# Autodesk Inventor assembly: TD6S-CHC_mockup
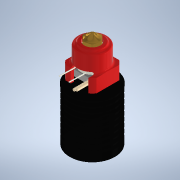
[picture p0: Inventor's stored thumbnail of the model, 180x180]
Saved by Autodesk Inventor 2020 (Build 240168000, 168)
## iProperties
Created: 2022-09-02
Part Number: TD6S-CHC_mockup
Description: STEP AP203
Document SubType Name: Assembly
Designer: Ishaan
Title: TD6S-CHC.STEP
Revision Number: ÈÎºÎ
## Documents named in this file (7)
- D:\Documents\Projects\Axiom - IDEX 3D Printer\CAD\00 - COTS Components\CHC Hotend\TD6S-CHC_mockup.iam
- D:\Documents\Projects\Axiom - IDEX 3D Printer\CAD\00 - COTS Components\CHC Hotend\Ã«Ï¸¹Üºí¹Ü×°Åä.iam
- D:\Documents\Projects\Axiom - IDEX 3D Printer\CAD\00 - COTS Components\CHC Hotend\»·ÐÎ¼ÓÈÈ¿é×°ÅäÌå1.iam
- D:\Documents\Projects\Axiom - IDEX 3D Printer\CAD\00 - COTS Components\CHC Hotend\socket head thin cap screw_din_DIN 7984 - M3 x 6 --- 4.5N.ipt
- D:\Documents\Projects\Axiom - IDEX 3D Printer\CAD\00 - COTS Components\CHC Hotend\»·ÐÎ¼ÓÈÈ¿é¹è½ºÌ×.ipt
- D:\Documents\Projects\Axiom - IDEX 3D Printer\CAD\00 - COTS Components\CHC Hotend\TV6-nozzle.ipt
- D:\Documents\Projects\Axiom - IDEX 3D Printer\CAD\00 - COTS Components\CHC Hotend\E3D-V6Ã«Ï¸¹Ü°æ±¾É¢ÈÈÆ÷-¦Õ16¹Ì¶¨¿×.ipt
## Components (6 placed, 6 different names)
1. Ã«Ï¸¹Üºí¹Ü×°Åä_1 [sub-assembly] — Mate:2
2. »·ÐÎ¼ÓÈÈ¿é×°ÅäÌå1_2 [sub-assembly]
3. socket head thin cap screw_din_DIN 7984 - M3 x 6 --- 4.5N_3 — Insert:1
4. »·ÐÎ¼ÓÈÈ¿é¹è½ºÌ×_4 — Mate:1, Angle:1
5. TV6-nozzle_5
6. E3D-V6Ã«Ï¸¹Ü°æ±¾É¢ÈÈÆ÷-¦Õ16¹Ì¶¨¿×_6 — Mate:1, Mate:2, Angle:1, Insert:1
## Relationships (4: Mate 2, Angle 1, Insert 1)
- Mate:1 (1.889 mm): »·ÐÎ¼ÓÈÈ¿é¹è½ºÌ×_4 ↔ E3D-V6Ã«Ï¸¹Ü°æ±¾É¢ÈÈÆ÷-¦Õ16¹Ì¶¨¿×_6
- Mate:2: Ã«Ï¸¹Üºí¹Ü×°Åä_1 ↔ E3D-V6Ã«Ï¸¹Ü°æ±¾É¢ÈÈÆ÷-¦Õ16¹Ì¶¨¿×_6
- Angle:1 (0 deg): »·ÐÎ¼ÓÈÈ¿é¹è½ºÌ×_4 ↔ E3D-V6Ã«Ï¸¹Ü°æ±¾É¢ÈÈÆ÷-¦Õ16¹Ì¶¨¿×_6
- Insert:1: socket head thin cap screw_din_DIN 7984 - M3 x 6 --- 4.5N_3 ↔ E3D-V6Ã«Ï¸¹Ü°æ±¾É¢ÈÈÆ÷-¦Õ16¹Ì¶¨¿×_6
